# Autodesk Inventor assembly: Mecanismo_base
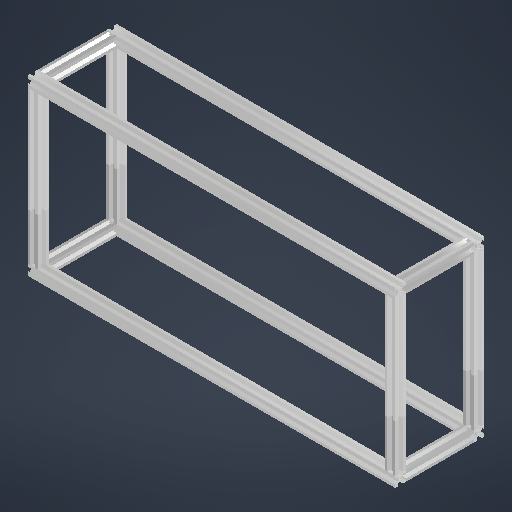
[picture p0: Inventor's stored thumbnail of the model, 512x512]
Saved by Autodesk Inventor 2026 (Build 300175050, 175E)
## iProperties
Created: 2025-10-12
Part Number: Mecanismo_base
Document SubType Name: Assembly
Designer: habbo
Author: habbo
## Documents named in this file (5)
- C:\Users\habbo\OneDrive\Documents\UTEC\2025-2\Mecanismo\Plataforma_validacion (1)\Plataforma_validacion\Mecanismo_base.iam
- C:\Users\habbo\OneDrive\Documents\UTEC\2025-2\Mecanismo\Plataforma_validacion (1)\Plataforma_validacion\vslot_700mm.ipt
- C:\Users\habbo\OneDrive\Documents\UTEC\2025-2\Mecanismo\Plataforma_validacion (1)\Plataforma_validacion\Plataforma_flotante\vslot_130mm.ipt
- C:\Users\habbo\OneDrive\Documents\UTEC\2025-2\Mecanismo\Plataforma_validacion (1)\Plataforma_validacion\Plataforma_flotante\vslot_200mm.ipt
- C:\Users\habbo\OneDrive\Documents\UTEC\2025-2\Mecanismo\Plataforma_validacion (1)\Plataforma_validacion\Plataforma_flotante\vslot_90mm.ipt
## Components (16 placed, 4 different names)
1. vslot_700mm:1 — Mate:10, Flush:21, Mate:11, Flush:22, Flush:33, Flush:34, Mate:18, Mate:19, Flush:38
2. vslot_700mm:2 — Flush:19, Flush:20, Flush:23, Mate:12, Flush:24, Flush:39, Flush:40, Mate:20, Flush:41, Flush:42, Mate:21
3. vslot_700mm:3 — Flush:1, Mate:1, Flush:2, Flush:6, Mate:17, Flush:35, Flush:36, Flush:37
4. vslot_700mm:4 — Flush:3, Mate:2, Flush:4, Flush:5, Mate:3
5. vslot_130mm:1 — Flush:5, Flush:6, Mate:3
6. vslot_130mm:2 — Flush:1, Mate:1, Flush:2, Flush:3, Mate:2, Flush:4
7. vslot_130mm:3 — Flush:19, Mate:10, Flush:20
8. vslot_130mm:4 — Flush:21, Mate:11, Flush:22, Flush:23, Mate:12, Flush:24
9. vslot_200mm:1 — Flush:25, Flush:26, Mate:13, Flush:41, Flush:42, Mate:21
10. vslot_200mm:2 — Flush:31, Flush:32, Mate:16, Flush:33, Flush:34, Mate:18
11. vslot_200mm:3 — Flush:27, Flush:28, Mate:14, Flush:37, Mate:19, Flush:38
12. vslot_200mm:4 — Mate:15, Flush:29, Flush:30, Flush:39, Flush:40, Mate:20
13. vslot_90mm:1 — Flush:25, Flush:26, Mate:13
14. vslot_90mm:2 — Flush:27, Flush:28, Mate:14
15. vslot_90mm:3 — Mate:15, Flush:29, Flush:30
16. vslot_90mm:4 — Flush:31, Flush:32, Mate:16, Mate:17, Flush:35, Flush:36
## Relationships (45: Flush 30, Mate 15)
- Flush:1: vslot_700mm:3 ↔ vslot_130mm:2
- Mate:1: vslot_700mm:3 ↔ vslot_130mm:2
- Flush:2: vslot_700mm:3 ↔ vslot_130mm:2
- Flush:3: vslot_700mm:4 ↔ vslot_130mm:2
- Mate:2: vslot_700mm:4 ↔ vslot_130mm:2
- Flush:4: vslot_700mm:4 ↔ vslot_130mm:2
- Flush:5: vslot_700mm:4 ↔ vslot_130mm:1
- Flush:6: vslot_700mm:3 ↔ vslot_130mm:1
- Mate:3: vslot_700mm:4 ↔ vslot_130mm:1
- Flush:19: vslot_700mm:2 ↔ vslot_130mm:3
- Mate:10: vslot_700mm:1 ↔ vslot_130mm:3
- Flush:20: vslot_700mm:2 ↔ vslot_130mm:3
- Flush:21: vslot_700mm:1 ↔ vslot_130mm:4
- Mate:11: vslot_700mm:1 ↔ vslot_130mm:4
- Flush:22: vslot_700mm:1 ↔ vslot_130mm:4
- Flush:23: vslot_700mm:2 ↔ vslot_130mm:4
- Mate:12: vslot_700mm:2 ↔ vslot_130mm:4
- Flush:24: vslot_700mm:2 ↔ vslot_130mm:4
- Flush:25: vslot_200mm:1 ↔ vslot_90mm:1
- Flush:26: vslot_200mm:1 ↔ vslot_90mm:1
- Mate:13: vslot_200mm:1 ↔ vslot_90mm:1
- Flush:27: vslot_200mm:3 ↔ vslot_90mm:2
- Flush:28: vslot_200mm:3 ↔ vslot_90mm:2
- Mate:14: vslot_200mm:3 ↔ vslot_90mm:2
- Mate:15: vslot_200mm:4 ↔ vslot_90mm:3
- Flush:29: vslot_200mm:4 ↔ vslot_90mm:3
- Flush:30: vslot_200mm:4 ↔ vslot_90mm:3
- Flush:31: vslot_200mm:2 ↔ vslot_90mm:4
- Flush:32: vslot_200mm:2 ↔ vslot_90mm:4
- Mate:16: vslot_200mm:2 ↔ vslot_90mm:4
- Flush:33: vslot_700mm:1 ↔ vslot_200mm:2
- Flush:34: vslot_700mm:1 ↔ vslot_200mm:2
- Mate:17: vslot_700mm:3 ↔ vslot_90mm:4
- Flush:35: vslot_700mm:3 ↔ vslot_90mm:4
- Flush:36: vslot_700mm:3 ↔ vslot_90mm:4
- Mate:18: vslot_700mm:1 ↔ vslot_200mm:2
- Flush:37: vslot_700mm:3 ↔ vslot_200mm:3
- Mate:19: vslot_700mm:1 ↔ vslot_200mm:3
- Flush:38: vslot_700mm:1 ↔ vslot_200mm:3
- Flush:39: vslot_700mm:2 ↔ vslot_200mm:4
- Flush:40: vslot_700mm:2 ↔ vslot_200mm:4
- Mate:20: vslot_700mm:2 ↔ vslot_200mm:4
- Flush:41: vslot_700mm:2 ↔ vslot_200mm:1
- Flush:42: vslot_700mm:2 ↔ vslot_200mm:1
- Mate:21: vslot_700mm:2 ↔ vslot_200mm:1
